# Autodesk Inventor assembly: gripper_assem
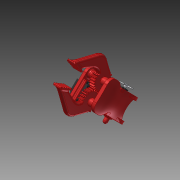
[picture p0: Inventor's stored thumbnail of the model, 180x180]
Saved by Autodesk Inventor 2014 (Build 180170000, 170)
## iProperties
Created: 2014-04-25
Part Number: gripper_assem
Document SubType Name: Assembly
Designer: t_emanb
Author: t_emanb
## Documents named in this file (8)
- C:\Users\t_emanb\Documents\3D printed arm\4th version\gripper_assem.iam
- C:\Users\t_emanb\Documents\3D printed arm\stock parts\microservo_assem.iam
- C:\Users\t_emanb\Documents\3D printed arm\4th version\upper_pin.ipt
- C:\Users\t_emanb\Documents\3D printed arm\4th version\upper_servo.ipt
- C:\Users\t_emanb\Documents\3D printed arm\4th version\gripper_gearMirror.ipt
- C:\Users\t_emanb\Documents\3D printed arm\4th version\gripper_base2.ipt
- C:\Users\t_emanb\Documents\3D printed arm\4th version\gripper_base.ipt
- C:\Users\t_emanb\Documents\3D printed arm\4th version\gripper_gearServo.ipt
## Components (8 placed, 6 different names)
1. upper_servo:1 — Mate:16, Flush:5, Mate:29, Mate:36, Mate:43, Mate:44
2. upper_pin:1 — Flush:1, Flush:2, Mate:17, Flush:3, Mate:26, Mate:35
3. Spur Gear1:2 — Mate:19, Mate:20
4. microservo_assem:2 [sub-assembly] — Mate:16, Mate:43, Mate:44
5. gripper_base2:1 — Flush:1, Flush:2, Mate:17, Mate:19, Mate:20, Mate:45, Mate:46, Mate:47
6. gripper_base:1 — Flush:3, Mate:26, Flush:5, Mate:29, Mate:35, Mate:36
7. Spur Gear1:3 — Mate:40, Mate:41, Mate:42
8. microservo_assem:3 [sub-assembly] — Mate:40, Mate:41, Mate:42, Mate:45, Mate:46, Mate:47
## Relationships (20: Mate 16, Flush 4)
- Mate:16: upper_servo:1 ↔ microservo_assem:2
- Flush:1: upper_pin:1 ↔ gripper_base2:1
- Flush:2: upper_pin:1 ↔ gripper_base2:1
- Mate:17: upper_pin:1 ↔ gripper_base2:1
- Mate:19: Spur Gear1:2 ↔ gripper_base2:1
- Mate:20: Spur Gear1:2 ↔ gripper_base2:1
- Flush:3: upper_pin:1 ↔ gripper_base:1
- Mate:26: upper_pin:1 ↔ gripper_base:1
- Flush:5: upper_servo:1 ↔ gripper_base:1
- Mate:29: upper_servo:1 ↔ gripper_base:1
- Mate:35: upper_pin:1 ↔ gripper_base:1
- Mate:36: upper_servo:1 ↔ gripper_base:1
- Mate:40: Spur Gear1:3 ↔ microservo_assem:3
- Mate:41: Spur Gear1:3 ↔ microservo_assem:3
- Mate:42: Spur Gear1:3 ↔ microservo_assem:3
- Mate:43: upper_servo:1 ↔ microservo_assem:2
- Mate:44: upper_servo:1 ↔ microservo_assem:2
- Mate:45: gripper_base2:1 ↔ microservo_assem:3
- Mate:46: gripper_base2:1 ↔ microservo_assem:3
- Mate:47: gripper_base2:1 ↔ microservo_assem:3
